# Autodesk Inventor assembly: Assembly5
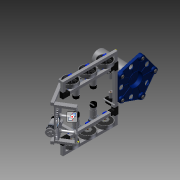
[picture p0: Inventor's stored thumbnail of the model, 180x180]
Saved by Autodesk Inventor 2015 (Build 190159000, 159)
## iProperties
Created: 2014-10-04
Part Number: Assembly5
Document SubType Name: Assembly
Designer: jesse
Author: jesse
## Documents named in this file (34)
- C:\Users\jesse\Desktop\robot\Assembly5.iam
- C:\Users\jesse\Desktop\robot\x base piece.ipt
- C:\Users\jesse\Desktop\robot\y base piece.ipt
- C:\Users\jesse\Desktop\robot\stock parts\am-2648_4inWheel8mmHub\am-2648_4inWheel8mmHub.iam
- C:\Users\jesse\Desktop\robot\stock parts\bronze_bushing_2012\bronze_bushing_2012.ipt
- C:\Users\jesse\Desktop\robot\inside wheel strut.ipt
- C:\Users\jesse\Desktop\robot\set of axle holders.iam
- C:\Users\jesse\Desktop\robot\stock parts\sprocket_25_24t_tetrix_2012\sprocket_25_24t_tetrix_2012.ipt
- C:\Users\jesse\Desktop\robot\stock parts\axle_d-shaft_2012\axle_d-shaft_2012.ipt
- C:\Users\jesse\Desktop\robot\stock parts\tetrix_739376_2pc_motormnt_2013\tetrix_739376_2pc_motormnt_2013-2.iam
- C:\Users\jesse\Desktop\robot\stock parts\am-2964NeveRest\am-2964NeveRest.ipt
- C:\Users\jesse\Desktop\robot\T clamp - bottom.ipt
- C:\Users\jesse\Desktop\robot\T clamp - top.ipt
- C:\Users\jesse\Desktop\robot\stock parts\hub_motor_shaft_2012\hub_motor_shaft_2012.ipt
- C:\Users\jesse\Desktop\robot\stock parts\axle_set_collar_2012\axle_set_collar_2012.ipt
- C:\Users\jesse\Desktop\robot\stock parts\screw_shcs_6-32_x_1_25_2012\screw_shcs_6-32_x_1_25_2012.ipt
- C:\Users\jesse\Desktop\robot\front peice.ipt
- C:\Users\jesse\Desktop\robot\arm\arm holder mount thing.ipt
- C:\Users\jesse\Desktop\robot\arm\sidepeices.ipt
- C:\Users\jesse\Desktop\robot\L clamp.iam
- C:\Users\jesse\Desktop\robot\flipper lift\flipper lift.iam
- C:\Users\jesse\Desktop\robot\arm\foam gripper.ipt
- C:\Users\jesse\Desktop\FTC_2014_2015_Field\2015_FTC_FOP_PTC\Imported Components\2015_ftc_fop_ptc\PENTAGON_GOAL_30.iam
- C:\Users\jesse\Desktop\robot\stock parts\servo_2012\servo_2012.iam
- C:\Users\jesse\Desktop\robot\rolling gripper\servo mount.ipt
- C:\Users\jesse\Desktop\robot\rolling gripper\goal holder.ipt
- C:\Users\jesse\Desktop\robot\axle holder.ipt
- C:\Users\jesse\Desktop\robot\rolling gripper\goal holder 2.ipt
- C:\Users\jesse\Desktop\robot\stock parts\3732-12_open_closed\3732-12_open_closed_04.ipt
- C:\Users\jesse\Desktop\robot\stock parts\3732-12_open_closed\3732-12_open_closed_05.ipt
- C:\Users\jesse\Desktop\robot\stock parts\3732-12_open_closed\3732-12_open_closed_01.ipt
- C:\Users\jesse\Desktop\robot\stock parts\3732-12_open_closed\3732-12_open_closed_02.ipt
- C:\Users\jesse\Desktop\robot\stock parts\3732-12_open_closed\3732-12_open_closed_03.ipt
- C:\Users\jesse\Desktop\robot\New Pickup\Assembly1.iam
## Components (116 placed, 33 different names)
1. x base piece:1 — Angle:7, Angle:8, Angle:9, Flush:34, Flush:35, Mate:73, Mate:242, Flush:242
2. y base piece:2 — Flush:6, Mate:3, Flush:34, Flush:35, Mate:73, Mate:74, Mate:75, Mate:76, Flush:36, Flush:37, Mate:101, Mate:102, Mate:104, Mate:105, Mate:281, Mate:282, Flush:259, Flush:260, Flush:261, Flush:262, Mate:288, Mate:289, Flush:263, Flush:265, Mate:301, Flush:266
3. x base piece:2 — Flush:6, Mate:3, Mate:32, Flush:12, Angle:1, Angle:2, Angle:3, Flush:18, Flush:19, Flush:20, Flush:37, Mate:239, Flush:112
4. am-2648_4inWheel8mmHub:8 [sub-assembly] — Mate:18, Mate:19, Mate:45, Mate:46, Mate:56, Mate:208, Mate:209, Mate:210, Mate:211, Mate:212
5. am-2648_4inWheel8mmHub:9 [sub-assembly] — Mate:20, Mate:21, Mate:43, Mate:44, Mate:57, Mate:213, Mate:214, Mate:215, Mate:216, Mate:217
6. am-2648_4inWheel8mmHub:10 [sub-assembly] — Mate:22, Mate:23, Mate:41, Mate:42, Mate:58, Mate:218, Mate:219, Mate:220, Mate:221, Mate:222
7. am-2648_4inWheel8mmHub:11 [sub-assembly] — Mate:16, Mate:17, Mate:50, Mate:51, Mate:54, Mate:202, Mate:203, Mate:204, Mate:205, Mate:206
8. am-2648_4inWheel8mmHub:12 [sub-assembly] — Mate:12, Mate:47, Mate:52, Mate:55, Mate:186, Mate:189, Mate:190, Mate:191, Mate:192, Mate:193, Mate:194, Mate:195, Mate:196
9. am-2648_4inWheel8mmHub:13 [sub-assembly] — Mate:14, Mate:15, Mate:48, Mate:49, Mate:53, Mate:197, Mate:198, Mate:199, Mate:200, Mate:201
10. bronze_bushing_2012:1 — Mate:12, Mate:186
11. bronze_bushing_2012:2 — Mate:14, Mate:15
12. bronze_bushing_2012:3 — Mate:16, Mate:17
13. bronze_bushing_2012:5 — Mate:20, Mate:21, Mate:34
14. bronze_bushing_2012:6 — Mate:22, Mate:23, Mate:35
15. bronze_bushing_2012:7 — Mate:18, Mate:19, Mate:33
16. inside wheel strut:1 — Mate:40, Flush:14, Angle:4, Angle:5, Angle:6, Mate:67, Mate:68, Angle:12, Angle:13, Mate:75, Mate:103, Flush:109, Flush:110, Mate:238, Flush:111, Flush:113, Mate:250, Flush:249, Mate:263
17. inside wheel strut:2 — Mate:39, Flush:15, Mate:65, Mate:66, Angle:10, Angle:11, Mate:74, Mate:76, Flush:36, Mate:106, Flush:107, Flush:108, Flush:241, Mate:241, Flush:243, Mate:252, Flush:250, Mate:258
18. set of axle holders:1 [sub-assembly] — Flush:13, Flush:16, Flush:21, Flush:22, Flush:23, Mate:188, Mate:234, Mate:236
19. set of axle holders:2 [sub-assembly] — Mate:32, Flush:12, Flush:13, Mate:33, Mate:34, Mate:35, Mate:59, Mate:60, Mate:61, Mate:227, Mate:230, Mate:232
20. set of axle holders:3 [sub-assembly] — Mate:40, Flush:14, Flush:17, Mate:77, Mate:265
21. set of axle holders:4 [sub-assembly] — Mate:39, Flush:15, Flush:16, Flush:17, Mate:62, Mate:63, Mate:64, Mate:264
22. sprocket_25_24t_tetrix_2012:1 — Mate:45, Mate:46, Mate:56, Rotation:4, Mate:88, Mate:89, Flush:246, Flush:247
23. sprocket_25_24t_tetrix_2012:2 — Mate:43, Mate:44, Mate:57, Rotation:3, Rotation:4, Mate:86, Flush:245, Flush:246
24. sprocket_25_24t_tetrix_2012:3 — Mate:41, Mate:42, Mate:58, Rotation:3, Mate:84, Mate:85, Flush:245, Flush:248
25. sprocket_25_24t_tetrix_2012:4 — Mate:47, Mate:52, Mate:55, Rotation:2, Mate:82, Mate:83, Flush:69, Flush:106
26. sprocket_25_24t_tetrix_2012:5 — Mate:48, Mate:49, Mate:53, Rotation:1, Rotation:2, Mate:80, Mate:81, Flush:105, Flush:251
27. sprocket_25_24t_tetrix_2012:6 — Mate:50, Mate:51, Mate:54, Rotation:1, Mate:78, Mate:79, Flush:252
28. axle_d-shaft_2012:1 — Mate:59, Angle:2, Angle:6, Flush:18, Mate:77, Mate:226
29. axle_d-shaft_2012:2 — Mate:64, Flush:21, Angle:7, Mate:233
30. axle_d-shaft_2012:3 — Mate:60, Angle:1, Angle:5, Flush:19, Mate:87, Mate:229
31. axle_d-shaft_2012:4 — Mate:61, Angle:3, Angle:4, Flush:20, Mate:231
32. axle_d-shaft_2012:5 — Mate:62, Angle:9, Flush:23, Mate:187
33. axle_d-shaft_2012:6 — Mate:63, Angle:8, Flush:22, Mate:235
34. tetrix_739376_2pc_motormnt_2013-2:1 [sub-assembly] — Mate:65, Mate:72, Flush:29, Flush:32, Flush:108
35. tetrix_739376_2pc_motormnt_2013-2:2 [sub-assembly] — Mate:66, Mate:69, Flush:28, Flush:33, Flush:107, Mate:253, Mate:264
36. tetrix_739376_2pc_motormnt_2013-2:3 [sub-assembly] — Mate:67, Mate:71, Flush:30, Flush:32, Flush:109, Mate:265
37. tetrix_739376_2pc_motormnt_2013-2:4 [sub-assembly] — Mate:68, Mate:70, Flush:31, Flush:33, Flush:110, Mate:251
38. am-2964NeveRest:1 — Mate:71, Flush:30, Angle:12, Mate:180
39. am-2964NeveRest:2 — Mate:69, Flush:28, Angle:11, Mate:182
40. am-2964NeveRest:3 — Mate:70, Flush:31, Angle:13, Mate:181
41. am-2964NeveRest:4 — Mate:72, Flush:29, Angle:10, Mate:183
42. bronze_bushing_2012:8 — Mate:78, Mate:79
43. bronze_bushing_2012:9 — Mate:80, Mate:81
44. bronze_bushing_2012:10 — Mate:82, Mate:83
45. bronze_bushing_2012:11 — Mate:84, Mate:85
46. bronze_bushing_2012:12 — Mate:86, Mate:87
47. bronze_bushing_2012:13 — Mate:88, Mate:89
48. T clamp - bottom:2 — Mate:104, Mate:105, Mate:106
49. T clamp - top:2
50. T clamp - bottom:4 — Mate:102
51. T clamp - top:4 — Mate:101, Mate:103
52. hub_motor_shaft_2012:1 — Mate:168, Mate:169, Mate:170, Mate:182
53. sprocket_25_24t_tetrix_2012:7 — Mate:168, Mate:169, Mate:170, Flush:251, Flush:252
54. hub_motor_shaft_2012:2 — Mate:183
55. sprocket_25_24t_tetrix_2012:8 — Flush:69, Flush:105, Flush:106
56. hub_motor_shaft_2012:3 — Mate:180
57. sprocket_25_24t_tetrix_2012:9 — Flush:247
58. hub_motor_shaft_2012:4
59. sprocket_25_24t_tetrix_2012:10 — Mate:181, Flush:248
60. axle_set_collar_2012:1 — Mate:187, Mate:188, Mate:237
61. screw_shcs_6-32_x_1_25_2012:1 — Mate:189, Mate:190
62. screw_shcs_6-32_x_1_25_2012:2 — Mate:191, Mate:192
63. screw_shcs_6-32_x_1_25_2012:3 — Mate:193, Mate:194
64. screw_shcs_6-32_x_1_25_2012:5 — Mate:195, Mate:196, Mate:237
65. screw_shcs_6-32_x_1_25_2012:6 — Flush:71, Mate:199
66. screw_shcs_6-32_x_1_25_2012:7 — Flush:72, Mate:198
67. screw_shcs_6-32_x_1_25_2012:8 — Flush:70, Flush:71, Mate:197, Mate:201
68. screw_shcs_6-32_x_1_25_2012:9 — Flush:70, Flush:72, Mate:200
69. screw_shcs_6-32_x_1_25_2012:14 — Mate:202
70. screw_shcs_6-32_x_1_25_2012:15 — Mate:204, Mate:206
71. screw_shcs_6-32_x_1_25_2012:16 — Mate:205
72. screw_shcs_6-32_x_1_25_2012:17 — Mate:203
73. screw_shcs_6-32_x_1_25_2012:18 — Mate:209, Mate:212
74. screw_shcs_6-32_x_1_25_2012:19 — Mate:210
75. screw_shcs_6-32_x_1_25_2012:20 — Mate:211
76. screw_shcs_6-32_x_1_25_2012:21 — Mate:208
77. screw_shcs_6-32_x_1_25_2012:22 — Mate:213, Mate:217
78. screw_shcs_6-32_x_1_25_2012:23 — Mate:214
79. screw_shcs_6-32_x_1_25_2012:24 — Mate:216
80. screw_shcs_6-32_x_1_25_2012:25 — Mate:215
81. screw_shcs_6-32_x_1_25_2012:26 — Mate:221
82. screw_shcs_6-32_x_1_25_2012:27 — Mate:219, Mate:222
83. screw_shcs_6-32_x_1_25_2012:28 — Mate:220, Mate:249
84. screw_shcs_6-32_x_1_25_2012:29 — Mate:218
85. axle_set_collar_2012:2 — Mate:226, Mate:227, Mate:249
86. axle_set_collar_2012:3 — Mate:229, Mate:230
87. axle_set_collar_2012:4 — Mate:231, Mate:232
88. axle_set_collar_2012:5 — Mate:233, Mate:234
89. axle_set_collar_2012:6 — Mate:235, Mate:236
90. front peice:1 — Mate:238, Mate:239, Flush:111, Flush:112, Flush:113, Mate:261, Mate:262
91. front peice:2 — Flush:241, Mate:241, Mate:242, Flush:242, Flush:243, Mate:259, Mate:260
92. arm holder mount thing:1 — Mate:250, Mate:251, Flush:249, Mate:254, Mate:255
93. arm holder mount thing:2 — Mate:252, Flush:250, Mate:253, Mate:256, Mate:257
94. sidepeices:1 — Mate:254, Mate:255, Flush:268
95. sidepeices:2 — Mate:256, Mate:257, Flush:268, Mate:315, Flush:269
96. L clamp:1 [sub-assembly] — Mate:258, Mate:259, Mate:260
97. L clamp:2 [sub-assembly] — Mate:261, Mate:262, Mate:263
98. flipper lift:1 [sub-assembly]
99. foam gripper:1
100. PENTAGON_GOAL_30:1 [sub-assembly] — Mate:281
101. servo_2012:1 [sub-assembly] — Mate:282, Flush:259, Mate:283, Mate:284, Mate:290, Mate:291, Mate:292
102. servo mount:1 — Flush:260, Flush:261, Flush:262, Mate:283, Mate:284
103. servo_2012:2 [sub-assembly] — Mate:287, Mate:303, Mate:304, Mate:305
104. servo mount:2 — Mate:287, Mate:288, Mate:289
105. goal holder:2 — Mate:290, Mate:291, Mate:292, Mate:298, Mate:299, Mate:302
106. bronze_bushing_2012:15 — Mate:298, Mate:299
107. axle holder:1 — Flush:263, Flush:265, Mate:308
108. axle holder:2 — Mate:301, Mate:302, Flush:266
109. goal holder 2:1 — Mate:303, Mate:304, Mate:305, Mate:306, Mate:307, Mate:308
110. bronze_bushing_2012:17 — Mate:306, Mate:307
111. 3732-12_open_closed_04:1 — Mate:309, Mate:310, Mate:311, Mate:312, Mate:313, Mate:314, Flush:267
112. 3732-12_open_closed_05:1
113. 3732-12_open_closed_01:1 — Mate:313, Mate:314, Flush:267
114. 3732-12_open_closed_02:1
115. 3732-12_open_closed_03:1 — Mate:309, Mate:310, Mate:311, Mate:312
116. Assembly1:1 [sub-assembly] — Mate:315, Flush:269
## Relationships (295: Mate 192, Flush 86, Angle 13, RelateRotation 4)
- Flush:6: y base piece:2 ↔ x base piece:2
- Mate:3: y base piece:2 ↔ x base piece:2
- [Mate]: x base piece:1 ↔ set of axle holders:1
- [Flush]: x base piece:1 ↔ set of axle holders:1
- [Mate]: am-2648_4inWheel8mmHub:12 ↔ set of axle holders:1
- [Mate]: am-2648_4inWheel8mmHub:13 ↔ set of axle holders:1
- [Mate]: am-2648_4inWheel8mmHub:11 ↔ set of axle holders:1
- Mate:12: am-2648_4inWheel8mmHub:12 ↔ bronze_bushing_2012:1
- Mate:14: am-2648_4inWheel8mmHub:13 ↔ bronze_bushing_2012:2
- Mate:15: am-2648_4inWheel8mmHub:13 ↔ bronze_bushing_2012:2
- Mate:16: am-2648_4inWheel8mmHub:11 ↔ bronze_bushing_2012:3
- Mate:17: am-2648_4inWheel8mmHub:11 ↔ bronze_bushing_2012:3
- Mate:18: am-2648_4inWheel8mmHub:8 ↔ bronze_bushing_2012:7
- Mate:19: am-2648_4inWheel8mmHub:8 ↔ bronze_bushing_2012:7
- Mate:20: am-2648_4inWheel8mmHub:9 ↔ bronze_bushing_2012:5
- Mate:21: am-2648_4inWheel8mmHub:9 ↔ bronze_bushing_2012:5
- Mate:22: am-2648_4inWheel8mmHub:10 ↔ bronze_bushing_2012:6
- Mate:23: am-2648_4inWheel8mmHub:10 ↔ bronze_bushing_2012:6
- Mate:32: x base piece:2 ↔ set of axle holders:2
- Flush:12: x base piece:2 ↔ set of axle holders:2
- Flush:13: set of axle holders:1 ↔ set of axle holders:2
- Mate:33: bronze_bushing_2012:7 ↔ set of axle holders:2
- Mate:34: bronze_bushing_2012:5 ↔ set of axle holders:2
- Mate:35: bronze_bushing_2012:6 ↔ set of axle holders:2
- Mate:39: inside wheel strut:2 ↔ set of axle holders:4
- Mate:40: inside wheel strut:1 ↔ set of axle holders:3
- Flush:14: inside wheel strut:1 ↔ set of axle holders:3
- Flush:15: inside wheel strut:2 ↔ set of axle holders:4
- Flush:16: set of axle holders:1 ↔ set of axle holders:4
- Flush:17: set of axle holders:3 ↔ set of axle holders:4
- Mate:41: am-2648_4inWheel8mmHub:10 ↔ sprocket_25_24t_tetrix_2012:3
- Mate:42: am-2648_4inWheel8mmHub:10 ↔ sprocket_25_24t_tetrix_2012:3
- Mate:43: am-2648_4inWheel8mmHub:9 ↔ sprocket_25_24t_tetrix_2012:2
- Mate:44: am-2648_4inWheel8mmHub:9 ↔ sprocket_25_24t_tetrix_2012:2
- Mate:45: am-2648_4inWheel8mmHub:8 ↔ sprocket_25_24t_tetrix_2012:1
- Mate:46: am-2648_4inWheel8mmHub:8 ↔ sprocket_25_24t_tetrix_2012:1
- Mate:47: am-2648_4inWheel8mmHub:12 ↔ sprocket_25_24t_tetrix_2012:4
- Mate:48: am-2648_4inWheel8mmHub:13 ↔ sprocket_25_24t_tetrix_2012:5
- Mate:49: am-2648_4inWheel8mmHub:13 ↔ sprocket_25_24t_tetrix_2012:5
- Mate:50: am-2648_4inWheel8mmHub:11 ↔ sprocket_25_24t_tetrix_2012:6
- Mate:51: am-2648_4inWheel8mmHub:11 ↔ sprocket_25_24t_tetrix_2012:6
- Mate:52: am-2648_4inWheel8mmHub:12 ↔ sprocket_25_24t_tetrix_2012:4
- Mate:53: am-2648_4inWheel8mmHub:13 ↔ sprocket_25_24t_tetrix_2012:5
- Mate:54: am-2648_4inWheel8mmHub:11 ↔ sprocket_25_24t_tetrix_2012:6
- Mate:55: am-2648_4inWheel8mmHub:12 ↔ sprocket_25_24t_tetrix_2012:4
- Mate:56: am-2648_4inWheel8mmHub:8 ↔ sprocket_25_24t_tetrix_2012:1
- Mate:57: am-2648_4inWheel8mmHub:9 ↔ sprocket_25_24t_tetrix_2012:2
- Mate:58: am-2648_4inWheel8mmHub:10 ↔ sprocket_25_24t_tetrix_2012:3
- Rotation:1 [RelateRotation] (1 ul): sprocket_25_24t_tetrix_2012:5 ↔ sprocket_25_24t_tetrix_2012:6
- Rotation:2 [RelateRotation] (1 ul): sprocket_25_24t_tetrix_2012:4 ↔ sprocket_25_24t_tetrix_2012:5
- Rotation:3 [RelateRotation] (1 ul): sprocket_25_24t_tetrix_2012:2 ↔ sprocket_25_24t_tetrix_2012:3
- Rotation:4 [RelateRotation] (1 ul): sprocket_25_24t_tetrix_2012:1 ↔ sprocket_25_24t_tetrix_2012:2
- Mate:59: set of axle holders:2 ↔ axle_d-shaft_2012:1
- Mate:60: set of axle holders:2 ↔ axle_d-shaft_2012:3
- Mate:61: set of axle holders:2 ↔ axle_d-shaft_2012:4
- Mate:62: set of axle holders:4 ↔ axle_d-shaft_2012:5
- Mate:63: set of axle holders:4 ↔ axle_d-shaft_2012:6
- Mate:64: set of axle holders:4 ↔ axle_d-shaft_2012:2
- Angle:1 (180 deg): x base piece:2 ↔ axle_d-shaft_2012:3
- Angle:2 (180 deg): x base piece:2 ↔ axle_d-shaft_2012:1
- Angle:3 (180 deg): x base piece:2 ↔ axle_d-shaft_2012:4
- Angle:4 (0 deg): inside wheel strut:1 ↔ axle_d-shaft_2012:4
- Angle:5 (0 deg): inside wheel strut:1 ↔ axle_d-shaft_2012:3
- Angle:6 (0 deg): inside wheel strut:1 ↔ axle_d-shaft_2012:1
- Flush:18: x base piece:2 ↔ axle_d-shaft_2012:1
- Flush:19: x base piece:2 ↔ axle_d-shaft_2012:3
- Flush:20: x base piece:2 ↔ axle_d-shaft_2012:4
- Flush:21: set of axle holders:1 ↔ axle_d-shaft_2012:2
- Angle:7 (0 deg): x base piece:1 ↔ axle_d-shaft_2012:2
- Angle:8 (0 deg): x base piece:1 ↔ axle_d-shaft_2012:6
- Angle:9 (0 deg): x base piece:1 ↔ axle_d-shaft_2012:5
- Flush:22: set of axle holders:1 ↔ axle_d-shaft_2012:6
- Flush:23: set of axle holders:1 ↔ axle_d-shaft_2012:5
- Mate:65: inside wheel strut:2 ↔ tetrix_739376_2pc_motormnt_2013-2:1
- Mate:66: inside wheel strut:2 ↔ tetrix_739376_2pc_motormnt_2013-2:2
- Mate:67: inside wheel strut:1 ↔ tetrix_739376_2pc_motormnt_2013-2:3
- Mate:68: inside wheel strut:1 ↔ tetrix_739376_2pc_motormnt_2013-2:4
- Mate:69: tetrix_739376_2pc_motormnt_2013-2:2 ↔ am-2964NeveRest:2
- Mate:70: tetrix_739376_2pc_motormnt_2013-2:4 ↔ am-2964NeveRest:3
- Mate:71: tetrix_739376_2pc_motormnt_2013-2:3 ↔ am-2964NeveRest:1
- Mate:72: tetrix_739376_2pc_motormnt_2013-2:1 ↔ am-2964NeveRest:4
- Flush:28: tetrix_739376_2pc_motormnt_2013-2:2 ↔ am-2964NeveRest:2
- Flush:29: tetrix_739376_2pc_motormnt_2013-2:1 ↔ am-2964NeveRest:4
- Flush:30: tetrix_739376_2pc_motormnt_2013-2:3 ↔ am-2964NeveRest:1
- Flush:31: tetrix_739376_2pc_motormnt_2013-2:4 ↔ am-2964NeveRest:3
- Flush:32: tetrix_739376_2pc_motormnt_2013-2:1 ↔ tetrix_739376_2pc_motormnt_2013-2:3
- Flush:33: tetrix_739376_2pc_motormnt_2013-2:2 ↔ tetrix_739376_2pc_motormnt_2013-2:4
- Angle:10 (90 deg): inside wheel strut:2 ↔ am-2964NeveRest:4
- Angle:11 (90 deg): inside wheel strut:2 ↔ am-2964NeveRest:2
- Angle:12 (-90 deg): inside wheel strut:1 ↔ am-2964NeveRest:1
- Angle:13 (90 deg): inside wheel strut:1 ↔ am-2964NeveRest:3
- Flush:34: x base piece:1 ↔ y base piece:2
- Flush:35: x base piece:1 ↔ y base piece:2
- Mate:73: x base piece:1 ↔ y base piece:2
- Mate:74: y base piece:2 ↔ inside wheel strut:2
- Mate:75: y base piece:2 ↔ inside wheel strut:1
- Mate:76: y base piece:2 ↔ inside wheel strut:2
- Flush:36: y base piece:2 ↔ inside wheel strut:2
- Mate:77: set of axle holders:3 ↔ axle_d-shaft_2012:1
- Flush:37: y base piece:2 ↔ x base piece:2
- Mate:78: sprocket_25_24t_tetrix_2012:6 ↔ bronze_bushing_2012:8
- Mate:79: sprocket_25_24t_tetrix_2012:6 ↔ bronze_bushing_2012:8
- Mate:80: sprocket_25_24t_tetrix_2012:5 ↔ bronze_bushing_2012:9
- Mate:81: sprocket_25_24t_tetrix_2012:5 ↔ bronze_bushing_2012:9
- Mate:82: sprocket_25_24t_tetrix_2012:4 ↔ bronze_bushing_2012:10
- Mate:83: sprocket_25_24t_tetrix_2012:4 ↔ bronze_bushing_2012:10
- Mate:84: sprocket_25_24t_tetrix_2012:3 ↔ bronze_bushing_2012:11
- Mate:85: sprocket_25_24t_tetrix_2012:3 ↔ bronze_bushing_2012:11
- Mate:86: sprocket_25_24t_tetrix_2012:2 ↔ bronze_bushing_2012:12
- Mate:87: axle_d-shaft_2012:3 ↔ bronze_bushing_2012:12
- Mate:88: sprocket_25_24t_tetrix_2012:1 ↔ bronze_bushing_2012:13
- Mate:89: sprocket_25_24t_tetrix_2012:1 ↔ bronze_bushing_2012:13
- [Flush]: T clamp - bottom:2 ↔ T clamp - top:2
- [Mate]: T clamp - bottom:2 ↔ T clamp - top:2
- [Flush]: T clamp - bottom:2 ↔ T clamp - top:2
- [Flush]: T clamp - bottom:4 ↔ T clamp - top:4
- [Mate]: T clamp - bottom:4 ↔ T clamp - top:4
- [Flush]: T clamp - bottom:4 ↔ T clamp - top:4
- Mate:101: y base piece:2 ↔ T clamp - top:4
- Mate:102: y base piece:2 ↔ T clamp - bottom:4
- Mate:103: inside wheel strut:1 ↔ T clamp - top:4
- Mate:104: y base piece:2 ↔ T clamp - bottom:2
- Mate:105: y base piece:2 ↔ T clamp - bottom:2
- Mate:106: inside wheel strut:2 ↔ T clamp - bottom:2
- Mate:168: hub_motor_shaft_2012:1 ↔ sprocket_25_24t_tetrix_2012:7
- Mate:169: hub_motor_shaft_2012:1 ↔ sprocket_25_24t_tetrix_2012:7
- Mate:170: hub_motor_shaft_2012:1 ↔ sprocket_25_24t_tetrix_2012:7
- [Mate]: hub_motor_shaft_2012:2 ↔ sprocket_25_24t_tetrix_2012:8
- [Mate]: hub_motor_shaft_2012:2 ↔ sprocket_25_24t_tetrix_2012:8
- [Mate]: hub_motor_shaft_2012:2 ↔ sprocket_25_24t_tetrix_2012:8
- [Mate]: hub_motor_shaft_2012:3 ↔ sprocket_25_24t_tetrix_2012:9
- [Mate]: hub_motor_shaft_2012:3 ↔ sprocket_25_24t_tetrix_2012:9
- [Mate]: hub_motor_shaft_2012:3 ↔ sprocket_25_24t_tetrix_2012:9
- [Mate]: hub_motor_shaft_2012:4 ↔ sprocket_25_24t_tetrix_2012:10
- [Mate]: hub_motor_shaft_2012:4 ↔ sprocket_25_24t_tetrix_2012:10
- [Mate]: hub_motor_shaft_2012:4 ↔ sprocket_25_24t_tetrix_2012:10
- Mate:180: am-2964NeveRest:1 ↔ hub_motor_shaft_2012:3
- Mate:181: am-2964NeveRest:3 ↔ sprocket_25_24t_tetrix_2012:10
- Mate:182: am-2964NeveRest:2 ↔ hub_motor_shaft_2012:1
- Mate:183: am-2964NeveRest:4 ↔ hub_motor_shaft_2012:2
- Flush:69: sprocket_25_24t_tetrix_2012:4 ↔ sprocket_25_24t_tetrix_2012:8
- Mate:186: am-2648_4inWheel8mmHub:12 ↔ bronze_bushing_2012:1
- Mate:187: axle_d-shaft_2012:5 ↔ axle_set_collar_2012:1
- Mate:188: set of axle holders:1 ↔ axle_set_collar_2012:1
- Mate:189: am-2648_4inWheel8mmHub:12 ↔ screw_shcs_6-32_x_1_25_2012:1
- Mate:190: am-2648_4inWheel8mmHub:12 ↔ screw_shcs_6-32_x_1_25_2012:1
- Mate:191: am-2648_4inWheel8mmHub:12 ↔ screw_shcs_6-32_x_1_25_2012:2
- Mate:192: am-2648_4inWheel8mmHub:12 ↔ screw_shcs_6-32_x_1_25_2012:2
- Mate:193: am-2648_4inWheel8mmHub:12 ↔ screw_shcs_6-32_x_1_25_2012:3
- Mate:194: am-2648_4inWheel8mmHub:12 ↔ screw_shcs_6-32_x_1_25_2012:3
- Mate:195: am-2648_4inWheel8mmHub:12 ↔ screw_shcs_6-32_x_1_25_2012:5
- Mate:196: am-2648_4inWheel8mmHub:12 ↔ screw_shcs_6-32_x_1_25_2012:5
- Flush:70: screw_shcs_6-32_x_1_25_2012:8 ↔ screw_shcs_6-32_x_1_25_2012:9
- Flush:71: screw_shcs_6-32_x_1_25_2012:6 ↔ screw_shcs_6-32_x_1_25_2012:8
- Flush:72: screw_shcs_6-32_x_1_25_2012:7 ↔ screw_shcs_6-32_x_1_25_2012:9
- Mate:197: am-2648_4inWheel8mmHub:13 ↔ screw_shcs_6-32_x_1_25_2012:8
- Mate:198: am-2648_4inWheel8mmHub:13 ↔ screw_shcs_6-32_x_1_25_2012:7
- Mate:199: am-2648_4inWheel8mmHub:13 ↔ screw_shcs_6-32_x_1_25_2012:6
- Mate:200: am-2648_4inWheel8mmHub:13 ↔ screw_shcs_6-32_x_1_25_2012:9
- Mate:201: am-2648_4inWheel8mmHub:13 ↔ screw_shcs_6-32_x_1_25_2012:8
- [Flush]: screw_shcs_6-32_x_1_25_2012:16 ↔ screw_shcs_6-32_x_1_25_2012:17
- [Flush]: screw_shcs_6-32_x_1_25_2012:14 ↔ screw_shcs_6-32_x_1_25_2012:16
- [Flush]: screw_shcs_6-32_x_1_25_2012:15 ↔ screw_shcs_6-32_x_1_25_2012:17
- [Flush]: screw_shcs_6-32_x_1_25_2012:14 ↔ screw_shcs_6-32_x_1_25_2012:17
- [Flush]: screw_shcs_6-32_x_1_25_2012:15 ↔ screw_shcs_6-32_x_1_25_2012:17
- [Flush]: screw_shcs_6-32_x_1_25_2012:14 ↔ screw_shcs_6-32_x_1_25_2012:16
- Mate:202: am-2648_4inWheel8mmHub:11 ↔ screw_shcs_6-32_x_1_25_2012:14
- Mate:203: am-2648_4inWheel8mmHub:11 ↔ screw_shcs_6-32_x_1_25_2012:17
- Mate:204: am-2648_4inWheel8mmHub:11 ↔ screw_shcs_6-32_x_1_25_2012:15
- Mate:205: am-2648_4inWheel8mmHub:11 ↔ screw_shcs_6-32_x_1_25_2012:16
- Mate:206: am-2648_4inWheel8mmHub:11 ↔ screw_shcs_6-32_x_1_25_2012:15
- [Flush]: screw_shcs_6-32_x_1_25_2012:20 ↔ screw_shcs_6-32_x_1_25_2012:21
- [Flush]: screw_shcs_6-32_x_1_25_2012:18 ↔ screw_shcs_6-32_x_1_25_2012:20
- [Flush]: screw_shcs_6-32_x_1_25_2012:19 ↔ screw_shcs_6-32_x_1_25_2012:21
- [Flush]: screw_shcs_6-32_x_1_25_2012:18 ↔ screw_shcs_6-32_x_1_25_2012:21
- [Flush]: screw_shcs_6-32_x_1_25_2012:19 ↔ screw_shcs_6-32_x_1_25_2012:21
- [Flush]: screw_shcs_6-32_x_1_25_2012:18 ↔ screw_shcs_6-32_x_1_25_2012:20
- Mate:208: am-2648_4inWheel8mmHub:8 ↔ screw_shcs_6-32_x_1_25_2012:21
- Mate:209: am-2648_4inWheel8mmHub:8 ↔ screw_shcs_6-32_x_1_25_2012:18
- Mate:210: am-2648_4inWheel8mmHub:8 ↔ screw_shcs_6-32_x_1_25_2012:19
- Mate:211: am-2648_4inWheel8mmHub:8 ↔ screw_shcs_6-32_x_1_25_2012:20
- Mate:212: am-2648_4inWheel8mmHub:8 ↔ screw_shcs_6-32_x_1_25_2012:18
- [Flush]: screw_shcs_6-32_x_1_25_2012:24 ↔ screw_shcs_6-32_x_1_25_2012:25
- [Flush]: screw_shcs_6-32_x_1_25_2012:22 ↔ screw_shcs_6-32_x_1_25_2012:24
- [Flush]: screw_shcs_6-32_x_1_25_2012:23 ↔ screw_shcs_6-32_x_1_25_2012:25
- [Flush]: screw_shcs_6-32_x_1_25_2012:22 ↔ screw_shcs_6-32_x_1_25_2012:25
- [Flush]: screw_shcs_6-32_x_1_25_2012:23 ↔ screw_shcs_6-32_x_1_25_2012:25
- [Flush]: screw_shcs_6-32_x_1_25_2012:22 ↔ screw_shcs_6-32_x_1_25_2012:24
- Mate:213: am-2648_4inWheel8mmHub:9 ↔ screw_shcs_6-32_x_1_25_2012:22
- Mate:214: am-2648_4inWheel8mmHub:9 ↔ screw_shcs_6-32_x_1_25_2012:23
- Mate:215: am-2648_4inWheel8mmHub:9 ↔ screw_shcs_6-32_x_1_25_2012:25
- Mate:216: am-2648_4inWheel8mmHub:9 ↔ screw_shcs_6-32_x_1_25_2012:24
- Mate:217: am-2648_4inWheel8mmHub:9 ↔ screw_shcs_6-32_x_1_25_2012:22
- [Flush]: screw_shcs_6-32_x_1_25_2012:28 ↔ screw_shcs_6-32_x_1_25_2012:29
- [Flush]: screw_shcs_6-32_x_1_25_2012:26 ↔ screw_shcs_6-32_x_1_25_2012:28
- [Flush]: screw_shcs_6-32_x_1_25_2012:27 ↔ screw_shcs_6-32_x_1_25_2012:29
- [Flush]: screw_shcs_6-32_x_1_25_2012:26 ↔ screw_shcs_6-32_x_1_25_2012:29
- [Flush]: screw_shcs_6-32_x_1_25_2012:27 ↔ screw_shcs_6-32_x_1_25_2012:29
- [Flush]: screw_shcs_6-32_x_1_25_2012:26 ↔ screw_shcs_6-32_x_1_25_2012:28
- Mate:218: am-2648_4inWheel8mmHub:10 ↔ screw_shcs_6-32_x_1_25_2012:29
- Mate:219: am-2648_4inWheel8mmHub:10 ↔ screw_shcs_6-32_x_1_25_2012:27
- Mate:220: am-2648_4inWheel8mmHub:10 ↔ screw_shcs_6-32_x_1_25_2012:28
- Mate:221: am-2648_4inWheel8mmHub:10 ↔ screw_shcs_6-32_x_1_25_2012:26
- Mate:222: am-2648_4inWheel8mmHub:10 ↔ screw_shcs_6-32_x_1_25_2012:27
- Mate:226: axle_d-shaft_2012:1 ↔ axle_set_collar_2012:2
- Mate:227: set of axle holders:2 ↔ axle_set_collar_2012:2
- Mate:229: axle_d-shaft_2012:3 ↔ axle_set_collar_2012:3
- Mate:230: set of axle holders:2 ↔ axle_set_collar_2012:3
- Mate:231: axle_d-shaft_2012:4 ↔ axle_set_collar_2012:4
- Mate:232: set of axle holders:2 ↔ axle_set_collar_2012:4
- Mate:233: axle_d-shaft_2012:2 ↔ axle_set_collar_2012:5
- Mate:234: set of axle holders:1 ↔ axle_set_collar_2012:5
- Flush:105: sprocket_25_24t_tetrix_2012:5 ↔ sprocket_25_24t_tetrix_2012:8
- Flush:106: sprocket_25_24t_tetrix_2012:4 ↔ sprocket_25_24t_tetrix_2012:8
- Mate:235: axle_d-shaft_2012:6 ↔ axle_set_collar_2012:6
- Mate:236: set of axle holders:1 ↔ axle_set_collar_2012:6
- Flush:107: inside wheel strut:2 ↔ tetrix_739376_2pc_motormnt_2013-2:2
- Flush:108: inside wheel strut:2 ↔ tetrix_739376_2pc_motormnt_2013-2:1
- Flush:109: inside wheel strut:1 ↔ tetrix_739376_2pc_motormnt_2013-2:3
- Flush:110: inside wheel strut:1 ↔ tetrix_739376_2pc_motormnt_2013-2:4
- Mate:237: axle_set_collar_2012:1 ↔ screw_shcs_6-32_x_1_25_2012:5
- Mate:238: inside wheel strut:1 ↔ front peice:1
- Mate:239: x base piece:2 ↔ front peice:1
- Flush:111: inside wheel strut:1 ↔ front peice:1
- Flush:112: x base piece:2 ↔ front peice:1
- Flush:113: inside wheel strut:1 ↔ front peice:1
- Flush:241: inside wheel strut:2 ↔ front peice:2
- Mate:241: inside wheel strut:2 ↔ front peice:2
- Mate:242: x base piece:1 ↔ front peice:2
- Flush:242: x base piece:1 ↔ front peice:2
- Flush:243: inside wheel strut:2 ↔ front peice:2
- Mate:249: screw_shcs_6-32_x_1_25_2012:28 ↔ axle_set_collar_2012:2
- Flush:245: sprocket_25_24t_tetrix_2012:2 ↔ sprocket_25_24t_tetrix_2012:3
- Flush:246: sprocket_25_24t_tetrix_2012:1 ↔ sprocket_25_24t_tetrix_2012:2
- Flush:247: sprocket_25_24t_tetrix_2012:1 ↔ sprocket_25_24t_tetrix_2012:9
- Flush:248: sprocket_25_24t_tetrix_2012:3 ↔ sprocket_25_24t_tetrix_2012:10
- Mate:250: inside wheel strut:1 ↔ arm holder mount thing:1
- Mate:251: tetrix_739376_2pc_motormnt_2013-2:4 ↔ arm holder mount thing:1
- Flush:249: inside wheel strut:1 ↔ arm holder mount thing:1
- Mate:252: inside wheel strut:2 ↔ arm holder mount thing:2
- Flush:250: inside wheel strut:2 ↔ arm holder mount thing:2
- Mate:253: tetrix_739376_2pc_motormnt_2013-2:2 ↔ arm holder mount thing:2
- Flush:251: sprocket_25_24t_tetrix_2012:5 ↔ sprocket_25_24t_tetrix_2012:7
- Flush:252: sprocket_25_24t_tetrix_2012:6 ↔ sprocket_25_24t_tetrix_2012:7
- Mate:254: arm holder mount thing:1 ↔ sidepeices:1
- Mate:255: arm holder mount thing:1 ↔ sidepeices:1
- Mate:256: arm holder mount thing:2 ↔ sidepeices:2
- Mate:257: arm holder mount thing:2 ↔ sidepeices:2
- Mate:258: inside wheel strut:2 ↔ L clamp:1
- Mate:259: front peice:2 ↔ L clamp:1
- Mate:260: front peice:2 ↔ L clamp:1
- Mate:261: front peice:1 ↔ L clamp:2
- Mate:262: front peice:1 ↔ L clamp:2
- Mate:263: inside wheel strut:1 ↔ L clamp:2
- Mate:264 (18.9992 mm): set of axle holders:4 ↔ tetrix_739376_2pc_motormnt_2013-2:2
- Mate:265 (18.9992 mm): set of axle holders:3 ↔ tetrix_739376_2pc_motormnt_2013-2:3
- Mate:281: y base piece:2 ↔ PENTAGON_GOAL_30:1
- Mate:282 (12.7 mm): y base piece:2 ↔ servo_2012:1
- Flush:259: y base piece:2 ↔ servo_2012:1
- Flush:260: y base piece:2 ↔ servo mount:1
- Flush:261: y base piece:2 ↔ servo mount:1
- Flush:262: y base piece:2 ↔ servo mount:1
- Mate:283: servo_2012:1 ↔ servo mount:1
- Mate:284: servo_2012:1 ↔ servo mount:1
- [Mate]: servo_2012:2 ↔ servo mount:2
- [Mate]: servo_2012:2 ↔ servo mount:2
- Mate:287: servo_2012:2 ↔ servo mount:2
- Mate:288: y base piece:2 ↔ servo mount:2
- Mate:289: y base piece:2 ↔ servo mount:2
- Mate:290: servo_2012:1 ↔ goal holder:2
- Mate:291: servo_2012:1 ↔ goal holder:2
- Mate:292: servo_2012:1 ↔ goal holder:2
- Mate:298: goal holder:2 ↔ bronze_bushing_2012:15
- Mate:299: goal holder:2 ↔ bronze_bushing_2012:15
- Flush:263: y base piece:2 ↔ axle holder:1
- Flush:265: y base piece:2 ↔ axle holder:1
- Mate:301: y base piece:2 ↔ axle holder:2
- Mate:302: goal holder:2 ↔ axle holder:2
- Flush:266: y base piece:2 ↔ axle holder:2
- Mate:303: servo_2012:2 ↔ goal holder 2:1
- Mate:304: servo_2012:2 ↔ goal holder 2:1
- Mate:305: servo_2012:2 ↔ goal holder 2:1
- Mate:306: goal holder 2:1 ↔ bronze_bushing_2012:17
- Mate:307: goal holder 2:1 ↔ bronze_bushing_2012:17
- Mate:308: axle holder:1 ↔ goal holder 2:1
- Mate:309 (-2.54 mm): 3732-12_open_closed_04:1 ↔ 3732-12_open_closed_03:1
- Mate:310 (-2.54 mm): 3732-12_open_closed_04:1 ↔ 3732-12_open_closed_03:1
- Mate:311 (-2.921 mm): 3732-12_open_closed_04:1 ↔ 3732-12_open_closed_03:1
- Mate:312 (158.8262 mm): 3732-12_open_closed_04:1 ↔ 3732-12_open_closed_03:1
- Mate:313 (5.08 mm): 3732-12_open_closed_04:1 ↔ 3732-12_open_closed_01:1
- Mate:314 (15.6972 mm): 3732-12_open_closed_04:1 ↔ 3732-12_open_closed_01:1
- Flush:267 (130.4544 mm): 3732-12_open_closed_04:1 ↔ 3732-12_open_closed_01:1
- Flush:268: sidepeices:1 ↔ sidepeices:2
- Mate:315: sidepeices:2 ↔ Assembly1:1
- Flush:269: sidepeices:2 ↔ Assembly1:1
## Named parameters: d171_d168 = 0 mm, d172_d169 = 0 mm, d173_d170 = 0 mm, d177_d168 = 0 mm, d178_d169 = 0 mm, d179_d170 = 0 mm, d288_d285 = 0 mm, d289_d286 = 0 mm, d290_d287 = 0 mm, d291_d285 = 0 mm, d292_d286 = 0 mm, d293_d287 = 0 mm, d294_d285 = 0 mm, d295_d286 = 0 mm, d296_d287 = 0 mm, d340_d334_d326 = 0 mm, d341_d335_d327 = 0 mm, d342_d336_d328 = 0 mm, d343_d337 = 0 mm, d344_d338 = 0 mm, d345_d339 = 0 mm, d352_d334_d326 = 0 mm, d353_d335_d327 = 0 mm, d354_d336_d328 = 0 mm, d355_d337 = 0 mm, d356_d338 = 0 mm, d357_d339 = 0 mm, d363_d334_d326 = 0 mm, d364_d335_d327 = 0 mm, d365_d336_d328 = 0 mm, d366_d337 = 0 mm, d367_d338 = 0 mm, d368_d339 = 0 mm, d374_d334_d326 = 0 mm, d375_d335_d327 = 0 mm, d376_d336_d328 = 0 mm, d377_d337 = 0 mm, d378_d338 = 0 mm, d379_d339 = 0 mm, d508_d506 = 0 mm, d509_d507 = 0 mm
